# Autodesk Inventor assembly: Transformador
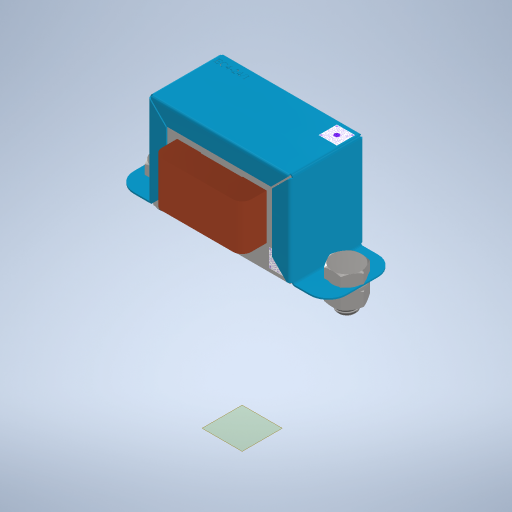
[picture p0: Inventor's stored thumbnail of the model, 512x512]
Saved by Autodesk Inventor 2024.2 (Build 282272000, 272)
## iProperties
Created: 2024-05-06
Part Number: Transformador
Document SubType Name: Assembly
Designer: 082220019
Author: 082220019
## Documents named in this file (8)
- C:\Users\082220019\Downloads\PBL-EC4-24-1-main (1)\PBL-EC4-24-1-main\Transformador.iam
- C:\Users\082220019\Downloads\PBL-EC4-24-1-main (1)\PBL-EC4-24-1-main\Fechamento.ipt
- C:\Users\082220019\Downloads\PBL-EC4-24-1-main (1)\PBL-EC4-24-1-main\Chapa.ipt
- C:\Users\082220019\Downloads\PBL-EC4-24-1-main (1)\PBL-EC4-24-1-main\Bobina.ipt
- C:\Users\082220019\Downloads\PBL-EC4-24-1-main (1)\PBL-EC4-24-1-main\Cobertura.ipt
- C:\Users\082220019\Documents\Inventor\Content Center Files\R2024\en-US\AS 1110\AS 1110 - M10 x 16.ipt
- C:\Users\082220019\Documents\Inventor\Content Center Files\R2024\en-US\AS 1237 (2.1)\AS 1237 - 10.ipt
- C:\Users\082220019\Documents\Inventor\Content Center Files\R2024\en-US\AS 1112 (2)\AS 1112 - M10  Type 5.ipt
## Components (218 placed, 7 different names)
1. Bobina:1
2. Cobertura:1 — Mate:2, Mate:3, Mate:4, Insert:1, Insert:2, Mate:6, Mate:8
3. AS 1110 - Metric M10 x 16:1 — Insert:1, Mate:7, Mate:11
4. AS 1110 - Metric M10 x 16:2 — Insert:2, Mate:5, Mate:9
5. AS 1237 (2.1) 10:1 — Mate:5, Mate:6, Mate:10
6. AS 1237 (2.1) 10:2 — Mate:7, Mate:8, Mate:12
7. AS 1112 (2) - Metric M10  Type 5:1 — Mate:9, Mate:10
8. AS 1112 (2) - Metric M10  Type 5:2 — Mate:11, Mate:12
9. Chapa:1 — Mate:1, Flush:1, Flush:2
10. Fechamento:1 — Mate:1, Flush:1, Flush:2
11. Chapa:2
12. Fechamento:2
13. Chapa:3
14. Fechamento:3
15. Chapa:4
16. Fechamento:4
17. Chapa:5
18. Fechamento:5
19. Chapa:6
20. Fechamento:6
21. Chapa:7
22. Fechamento:7
23. Chapa:8
24. Fechamento:8
25. Chapa:9
26. Fechamento:9
27. Chapa:10
28. Fechamento:10
29. Chapa:11
30. Fechamento:11
31. Chapa:12
32. Fechamento:12
33. Chapa:13
34. Fechamento:13
35. Chapa:14
36. Fechamento:14
37. Chapa:15
38. Fechamento:15
39. Chapa:16
40. Fechamento:16
41. Chapa:17
42. Fechamento:17
43. Chapa:18
44. Fechamento:18
45. Chapa:19
46. Fechamento:19
47. Chapa:20
48. Fechamento:20
49. Chapa:21
50. Fechamento:21
51. Chapa:22
52. Fechamento:22
53. Chapa:23
54. Fechamento:23
55. Chapa:24
56. Fechamento:24
57. Chapa:25
58. Fechamento:25
59. Chapa:26
60. Fechamento:26
61. Chapa:27
62. Fechamento:27
63. Chapa:28
64. Fechamento:28
65. Chapa:29
66. Fechamento:29
67. Chapa:30
68. Fechamento:30
69. Chapa:31
70. Fechamento:31
71. Chapa:32
72. Fechamento:32
73. Chapa:33
74. Fechamento:33
75. Chapa:34
76. Fechamento:34
77. Chapa:35
78. Fechamento:35
79. Chapa:36
80. Fechamento:36
81. Chapa:37
82. Fechamento:37
83. Chapa:38
84. Fechamento:38
85. Chapa:39
86. Fechamento:39
87. Chapa:40
88. Fechamento:40
89. Chapa:41
90. Fechamento:41
91. Chapa:42
92. Fechamento:42
93. Chapa:43
94. Fechamento:43
95. Chapa:44
96. Fechamento:44
97. Chapa:45
98. Fechamento:45
99. Chapa:46
100. Fechamento:46
101. Chapa:47
102. Fechamento:47
103. Chapa:48
104. Fechamento:48
105. Chapa:49
106. Fechamento:49
107. Chapa:50
108. Fechamento:50
109. Chapa:51
110. Fechamento:51
111. Chapa:52
112. Fechamento:52
113. Chapa:53
114. Fechamento:53
115. Chapa:54
116. Fechamento:54
117. Chapa:55
118. Fechamento:55
119. Chapa:56
120. Fechamento:56
121. Chapa:57
122. Fechamento:57
123. Chapa:58
124. Fechamento:58
125. Chapa:59
126. Fechamento:59
127. Chapa:60
128. Fechamento:60
129. Chapa:61
130. Fechamento:61
131. Chapa:62
132. Fechamento:62
133. Chapa:63
134. Fechamento:63
135. Chapa:64
136. Fechamento:64
137. Chapa:65
138. Fechamento:65
139. Chapa:66
140. Fechamento:66
141. Chapa:67
142. Fechamento:67
143. Chapa:68
144. Fechamento:68
145. Chapa:69
146. Fechamento:69
147. Chapa:70
148. Fechamento:70 — Mate:3
149. Chapa:71
150. Fechamento:71
151. Chapa:72
152. Fechamento:72
153. Chapa:73
154. Fechamento:73
155. Chapa:74
156. Fechamento:74
157. Chapa:75
158. Fechamento:75
159. Chapa:76
160. Fechamento:76
161. Chapa:77
162. Fechamento:77
163. Chapa:78
164. Fechamento:78
165. Chapa:79
166. Fechamento:79
167. Chapa:80
168. Fechamento:80
169. Chapa:81
170. Fechamento:81
171. Chapa:82
172. Fechamento:82
173. Chapa:83
174. Fechamento:83
175. Chapa:84
176. Fechamento:84
177. Chapa:85 — Mate:4
178. Fechamento:85
179. Chapa:86
180. Fechamento:86
181. Chapa:87
182. Fechamento:87
183. Chapa:88
184. Fechamento:88
185. Chapa:89
186. Fechamento:89
187. Chapa:90
188. Fechamento:90
189. Chapa:91
190. Fechamento:91
191. Chapa:92
192. Fechamento:92
193. Chapa:93
194. Fechamento:93
195. Chapa:94
196. Fechamento:94
197. Chapa:95
198. Fechamento:95
199. Chapa:96
200. Fechamento:96
201. Chapa:97
202. Fechamento:97
203. Chapa:98
204. Fechamento:98
205. Chapa:99
206. Fechamento:99
207. Chapa:100
208. Fechamento:100
209. Chapa:101
210. Fechamento:101
211. Chapa:102
212. Fechamento:102
213. Chapa:103
214. Fechamento:103
215. Chapa:104
216. Fechamento:104
217. Chapa:105 — Mate:2
218. Fechamento:105
## Component patterns: (105 elements, first: Chapa:1 + Fechamento:1)
## Relationships (16: Mate 12, Flush 2, Insert 2)
- Mate:1: Chapa:1 ↔ Fechamento:1
- Flush:1: Chapa:1 ↔ Fechamento:1
- Flush:2: Chapa:1 ↔ Fechamento:1
- Mate:2 (0.8 mm): Cobertura:1 ↔ Chapa:105
- Mate:3 (0.8 mm): Cobertura:1 ↔ Fechamento:70
- Mate:4 (0.8 mm): Cobertura:1 ↔ Chapa:85
- Insert:1: Cobertura:1 ↔ AS 1110 - Metric M10 x 16:1
- Insert:2: Cobertura:1 ↔ AS 1110 - Metric M10 x 16:2
- Mate:5: AS 1110 - Metric M10 x 16:2 ↔ AS 1237 (2.1) 10:1
- Mate:6: Cobertura:1 ↔ AS 1237 (2.1) 10:1
- Mate:7: AS 1110 - Metric M10 x 16:1 ↔ AS 1237 (2.1) 10:2
- Mate:8: Cobertura:1 ↔ AS 1237 (2.1) 10:2
- Mate:9: AS 1110 - Metric M10 x 16:2 ↔ AS 1112 (2) - Metric M10  Type 5:1
- Mate:10: AS 1237 (2.1) 10:1 ↔ AS 1112 (2) - Metric M10  Type 5:1
- Mate:11: AS 1110 - Metric M10 x 16:1 ↔ AS 1112 (2) - Metric M10  Type 5:2
- Mate:12: AS 1237 (2.1) 10:2 ↔ AS 1112 (2) - Metric M10  Type 5:2
